# Autodesk Inventor assembly: sensorBoard
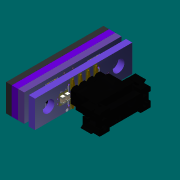
[picture p0: Inventor's stored thumbnail of the model, 180x180]
Saved by Autodesk Inventor 2016 SP1 (Build 200210100, 210)
## iProperties
Created: 2016-02-15
Part Number: sensorBoard
Document SubType Name: Assembly
Designer: sawai
Author: sawai
## Documents named in this file (8)
- C:\Users\sawaiz\OneDrive\projects\mppcSensor\cad\mppcSensor.iam
- C:\Users\sawaiz\oneDrive\projects\mppcSensor\cad\sensorBoardA\pcb.ipt
- C:\Users\sawaiz\oneDrive\projects\mppcSensor\cad\sensorBoardB\boardB.iam
- C:\Users\sawaiz\oneDrive\projects\mppcSensor\cad\sensorBoardC\boardC.iam
- C:\Users\sawaiz\oneDrive\projects\mppcSensor\cad\sensorBoardA\groundGlassDisc.ipt
- C:\Users\sawaiz\oneDrive\projects\mppcSensor\cad\sensorBoardA\lightGasket.ipt
- C:\Users\sawaiz\oneDrive\projects\mppcSensor\cad\electronics\2x4header.ipt
- C:\Users\sawaiz\oneDrive\projects\mppcSensor\cad\electronics\2x4RibbonConnector.ipt
## Components (7 placed, 7 different names)
1. pcb:1 — Flush:3, Flush:4, Mate:1, Flush:6, Flush:7, Mate:3, Mate:4
2. boardB:1 [sub-assembly] — Flush:1, Flush:2, Flush:3, Flush:4, Mate:2, Mate:3
3. boardC:1 [sub-assembly] — Flush:1, Flush:2, Mate:2, Mate:6, Angle:1, Angle:2, Angle:3
4. groundGlassDisc:1 — Mate:1, Flush:8
5. lightGasket:1 — Flush:6, Flush:7, Mate:4, Flush:8
6. 2x4header:1 — Mate:6, Angle:1, Mate:7, Mate:8, Mate:9
7. 2x4RibbonConnector:1 — Angle:2, Angle:3, Mate:7, Mate:8, Mate:9
## Relationships (18: Mate 8, Flush 7, Angle 3)
- Flush:1: boardB:1 ↔ boardC:1
- Flush:2: boardB:1 ↔ boardC:1
- Flush:3: pcb:1 ↔ boardB:1
- Flush:4: pcb:1 ↔ boardB:1
- Mate:1: pcb:1 ↔ groundGlassDisc:1
- Flush:6: pcb:1 ↔ lightGasket:1
- Flush:7: pcb:1 ↔ lightGasket:1
- Mate:2: boardB:1 ↔ boardC:1
- Mate:3: pcb:1 ↔ boardB:1
- Mate:4: pcb:1 ↔ lightGasket:1
- Mate:6: boardC:1 ↔ 2x4header:1
- Angle:1 (0 deg): boardC:1 ↔ 2x4header:1
- Angle:2 (0 deg): boardC:1 ↔ 2x4RibbonConnector:1
- Angle:3 (0 deg): boardC:1 ↔ 2x4RibbonConnector:1
- Mate:7 (0.05 mm): 2x4header:1 ↔ 2x4RibbonConnector:1
- Mate:8 (0.05 mm): 2x4header:1 ↔ 2x4RibbonConnector:1
- Mate:9: 2x4header:1 ↔ 2x4RibbonConnector:1
- Flush:8: groundGlassDisc:1 ↔ lightGasket:1
